# Autodesk Inventor assembly: Pool House 02
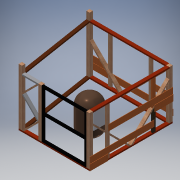
[picture p0: Inventor's stored thumbnail of the model, 180x180]
Saved by Autodesk Inventor 2016 (Build 200138000, 138)
## iProperties
Created: 2015-05-30
Part Number: Pool House 02
Document SubType Name: Assembly
Designer: steele
Author: steele
## Documents named in this file (28)
- C:\snobotics\CAD-Development\robSteele\HouseProjects\PoolHouseProject\Pool House 02.iam
- C:\snobotics\CAD-Development\robSteele\HouseProjects\PoolHouseProject\Base for Pool House.ipt
- C:\snobotics\CAD-Development\robSteele\HouseProjects\PoolHouseProject\Front Post North Side.ipt
- C:\snobotics\CAD-Development\robSteele\HouseProjects\PoolHouseProject\Front Post South Side.ipt
- C:\snobotics\CAD-Development\robSteele\HouseProjects\PoolHouseProject\Rear Post South Side.ipt
- C:\snobotics\CAD-Development\robSteele\HouseProjects\PoolHouseProject\Pool Controller.ipt
- C:\snobotics\CAD-Development\robSteele\HouseProjects\PoolHouseProject\Home Depot Composite Slat 69 in.ipt
- C:\snobotics\CAD-Development\robSteele\HouseProjects\PoolHouseProject\Home Depot Composite Slat 19_75 in.ipt
- C:\snobotics\CAD-Development\robSteele\HouseProjects\PoolHouseProject\Lumber 2x4x82.ipt
- C:\snobotics\CAD-Development\robSteele\HouseProjects\PoolHouseProject\Lumbwer 2x4x50_75.ipt
- C:\snobotics\CAD-Development\robSteele\HouseProjects\PoolHouseProject\Lumber 2x4x80.ipt
- C:\snobotics\CAD-Development\robSteele\HouseProjects\PoolHouseProject\Pool Filter.ipt
- C:\snobotics\CAD-Development\robSteele\HouseProjects\PoolHouseProject\Pool Door.ipt
- C:\snobotics\CAD-Development\robSteele\HouseProjects\PoolHouseProject\58 Inch 45 Diagonal Piece.ipt
- C:\snobotics\CAD-Development\robSteele\HouseProjects\PoolHouseProject\Roof.ipt
- C:\snobotics\CAD-Development\robSteele\HouseProjects\PoolHouseProject\Front Face Bottom Support for Slats.ipt
- C:\snobotics\CAD-Development\robSteele\HouseProjects\PoolHouseProject\Front Face Upper Support for Slats.ipt
- C:\snobotics\CAD-Development\robSteele\HouseProjects\PoolHouseProject\Right Panel Rear 45 Diagonal Piece.ipt
- C:\snobotics\CAD-Development\robSteele\HouseProjects\PoolHouseProject\New Rear Post North Side.ipt
- C:\snobotics\CAD-Development\robSteele\HouseProjects\PoolHouseProject\Right Panel Front 45 Diagonal Piece.ipt
- C:\snobotics\CAD-Development\robSteele\HouseProjects\PoolHouseProject\Back 2x4.ipt
- C:\snobotics\CAD-Development\robSteele\HouseProjects\PoolHouseProject\Support 2x4.ipt
- C:\snobotics\CAD-Development\robSteele\HouseProjects\PoolHouseProject\Home Depot Composite Slat 51_5 in.ipt
- C:\snobotics\CAD-Development\robSteele\HouseProjects\PoolHouseProject\2x4 17.5 Inch.ipt
- C:\snobotics\CAD-Development\robSteele\HouseProjects\PoolHouseProject\Short Wall 45 Diagonal Piece.ipt
- C:\snobotics\CAD-Development\robSteele\HouseProjects\PoolHouseProject\Home Depot Composite Slat 24_50 in.ipt
- C:\snobotics\CAD-Development\robSteele\HouseProjects\PoolHouseProject\Home Depot Composite Slat 23 in.ipt
- C:\snobotics\CAD-Development\robSteele\HouseProjects\PoolHouseProject\Home Depot Composite Slat 66 3_16 in.ipt
## Components (76 placed, 27 different names)
1. Base for Pool House:1 — Mate:1, Flush:1, Flush:2, Mate:2, Flush:3, Flush:4, Mate:3, Flush:5, Flush:6, Mate:4, Flush:7, Flush:8, Mate:8, Flush:11, Mate:9, Mate:10, Flush:21, Flush:22, Mate:77, Mate:79, Mate:82, Flush:32, Mate:84, Flush:33, Flush:34, Tangent:1, Tangent:2, Mate:93, Mate:100, Mate:102, Mate:112, Mate:114, Mate:115, Flush:47, Flush:48, Mate:116, Flush:49, Mate:117, Mate:119, Mate:127
2. Front Post North Side:1 — Mate:1, Flush:1, Flush:2, Mate:5, Flush:9, Flush:10, Mate:11, Mate:12, Mate:13, Mate:20, Mate:24, Mate:28, Mate:32, Mate:38, Mate:40, Mate:78, Flush:58, Flush:59, Flush:60, Flush:73
3. Front Post South Side:1 — Mate:2, Flush:3, Flush:4, Mate:7, Mate:15, Mate:22, Mate:27, Mate:30, Mate:34, Mate:36, Mate:42, Mate:80, Mate:81, Flush:30, Flush:31, Mate:85, Mate:94, Flush:38, Mate:101, Flush:40, Mate:104, Mate:108, Mate:111, Flush:45, Flush:74
4. Front Post North Side:3 — Mate:3, Flush:5, Flush:6, Mate:92, Mate:118, Flush:50, Flush:51, Mate:120
5. Rear Post South Side:1 — Mate:4, Flush:7, Flush:8, Mate:45, Mate:47, Mate:53, Mate:55, Mate:61, Mate:69, Mate:71, Mate:75, Mate:83, Mate:113, Flush:46
6. Pool Controller:1 — Mate:5, Flush:9, Flush:10
7. Lumber 2x4x82:1 — Mate:11, Mate:12, Mate:97
8. Home Depot Composite Slat 69 in:1 — Mate:7, Mate:8, Flush:11, Mate:16, Flush:14, Mate:46, Flush:61
9. Home Depot Composite Slat 19_75 in:1 — Mate:9, Mate:10, Mate:14, Flush:14
10. Home Depot Composite Slat 69 in:2 — Mate:13, Mate:14, Mate:21, Mate:23, Flush:13, Flush:60
11. Home Depot Composite Slat 19_75 in:2 — Mate:15, Mate:16, Flush:13, Mate:49
12. Home Depot Composite Slat 69 in:3 — Mate:22, Mate:23, Flush:12, Mate:26, Mate:51, Flush:62
13. Home Depot Composite Slat 19_75 in:3 — Mate:20, Mate:21, Flush:12, Mate:25
14. Home Depot Composite Slat 69 in:4 — Mate:24, Mate:25, Flush:15, Mate:29, Flush:59
15. Home Depot Composite Slat 19_75 in:4 — Mate:26, Mate:27, Flush:15, Mate:31, Mate:57
16. Home Depot Composite Slat 19_75 in:5 — Mate:28, Mate:29, Flush:16
17. Home Depot Composite Slat 69 in:5 — Mate:30, Mate:31, Flush:16, Mate:33, Mate:35, Mate:59, Flush:63
18. Home Depot Composite Slat 69 in:6 — Mate:32, Mate:33, Flush:17, Mate:39
19. Home Depot Composite Slat 19_75 in:6 — Mate:34, Mate:35, Flush:17, Mate:37, Flush:29, Flush:64
20. Home Depot Composite Slat 69 in:7 — Mate:36, Mate:37, Flush:18, Mate:41, Mate:43, Mate:65, Flush:29, Flush:65
21. Home Depot Composite Slat 19_75 in:7 — Mate:38, Mate:39, Flush:18
22. Home Depot Composite Slat 69 in:8 — Mate:40, Mate:41, Flush:19, Mate:148, Flush:58
23. Home Depot Composite Slat 19_75 in:8 — Mate:42, Mate:43, Flush:19, Mate:67, Mate:73
24. Home Depot Composite Slat 23 in:1 — Mate:45, Flush:21, Mate:48, Flush:23
25. Home Depot Composite Slat 66 3_16 in:1 — Mate:46, Flush:22, Flush:23, Mate:50, Flush:61
26. Home Depot Composite Slat 66 3_16 in:2 — Mate:47, Mate:48, Flush:24, Mate:54
27. Home Depot Composite Slat 23 in:8 — Mate:49, Mate:50, Flush:24, Mate:52
28. Home Depot Composite Slat 66 3_16 in:3 — Mate:51, Mate:52, Flush:25, Mate:58, Flush:62
29. Home Depot Composite Slat 23 in:4 — Mate:53, Mate:54, Flush:25, Mate:56
30. Home Depot Composite Slat 66 3_16 in:8 — Mate:55, Mate:56, Flush:26, Mate:62
31. Home Depot Composite Slat 23 in:5 — Mate:57, Mate:58, Flush:26, Mate:60
32. Home Depot Composite Slat 66 3_16 in:7 — Mate:59, Mate:60, Flush:27, Mate:64, Mate:70, Flush:63
33. Home Depot Composite Slat 66 3_16 in:5 — Mate:64, Mate:69, Flush:28, Mate:72
34. Home Depot Composite Slat 66 3_16 in:6 — Mate:67, Mate:68, Mate:74, Mate:76, Flush:65
35. Home Depot Composite Slat 23 in:2 — Mate:61, Mate:62, Flush:27
36. Home Depot Composite Slat 23 in:6 — Mate:65, Mate:68, Mate:70, Flush:28, Flush:64
37. Home Depot Composite Slat 23 in:7 — Mate:71, Mate:72
38. Home Depot Composite Slat 23 in:3 — Mate:73, Mate:74, Mate:151
39. Home Depot Composite Slat 66 3_16 in:4 — Mate:75, Mate:76
40. Lumbwer 2x4x50_75:1 — Mate:77, Mate:78, Mate:148
41. Lumbwer 2x4x50_75:2 — Mate:79, Mate:80
42. Lumber 2x4x80:1 — Mate:81, Flush:30, Flush:31
43. Lumbwer 2x4x50_75:3 — Mate:82, Mate:83, Flush:32
44. Lumbwer 2x4x50_75:4 — Mate:84, Mate:85, Flush:33, Mate:151
45. Pool Filter:1 — Flush:34, Tangent:1, Tangent:2
46. Pool Door:1 — Mate:92, Mate:93, Mate:146, Mate:147, Flush:57, Mate:153, Flush:66, Mate:155, Flush:67, Mate:157, Flush:68, Mate:159, Flush:69, Mate:161, Flush:70, Mate:163, Flush:71, Mate:165, Flush:72
47. 58 Inch 45 Diagonal Piece:1 — Mate:100, Flush:73
48. 58 Inch 45 Diagonal Piece:2 — Mate:94, Flush:38, Mate:97, Mate:101, Mate:102, Flush:40, Mate:103, Flush:41, Mate:107, Flush:42, Flush:74
49. Roof:1
50. Front Face Bottom Support for Slats:1 — Mate:103, Mate:104, Flush:41
51. Front Face Upper Support for Slats:2 — Mate:107, Mate:108, Flush:42
52. Right Panel Front 45 Diagonal Piece:1 — Mate:111, Mate:112, Flush:45
53. Right Panel Rear 45 Diagonal Piece:2 — Mate:113, Mate:114, Flush:46
54. New Rear Post North Side:1 — Mate:115, Flush:47, Flush:48, Flush:52, Mate:122, Flush:53, Mate:123, Mate:124, Mate:128, Mate:129, Mate:132, Mate:133, Mate:134, Mate:136, Mate:138, Mate:140, Mate:142
55. Back 2x4:1 — Mate:116, Flush:49, Mate:117
56. 2x4 17.5 Inch:1 — Mate:118, Flush:50, Flush:51, Mate:121, Flush:54
57. Short Wall 45 Diagonal Piece:2 — Mate:119, Mate:120, Flush:52
58. Short Wall 45 Diagonal Piece:1 — Mate:121, Mate:122, Flush:53, Flush:56, Mate:149, Mate:150
59. Back 2x4:2 — Mate:123, Flush:54, Mate:124
60. Home Depot Composite Slat 24_50 in:1 — Mate:127, Mate:128, Mate:130
61. Home Depot Composite Slat 24_50 in:2 — Mate:129, Mate:130, Mate:131
62. Home Depot Composite Slat 24_50 in:3 — Mate:131, Mate:132, Mate:135
63. Home Depot Composite Slat 24_50 in:4 — Mate:133, Mate:134, Mate:135, Mate:137
64. Home Depot Composite Slat 24_50 in:5 — Mate:136, Mate:137, Mate:139
65. Home Depot Composite Slat 24_50 in:6 — Mate:138, Mate:139, Mate:141
66. Home Depot Composite Slat 24_50 in:7 — Mate:140, Mate:141, Mate:143
67. Home Depot Composite Slat 24_50 in:8 — Mate:142, Mate:143
68. Support 2x4:1 — Flush:56, Mate:149, Mate:150
69. Home Depot Composite Slat 51_5 in:1 — Mate:146, Mate:147, Flush:57, Mate:152
70. Home Depot Composite Slat 51_5 in:2 — Mate:152, Mate:153, Flush:66, Mate:154
71. Home Depot Composite Slat 51_5 in:3 — Mate:154, Mate:155, Flush:67, Mate:156
72. Home Depot Composite Slat 51_5 in:4 — Mate:156, Mate:157, Flush:68, Mate:158
73. Home Depot Composite Slat 51_5 in:5 — Mate:158, Mate:159, Flush:69, Mate:160
74. Home Depot Composite Slat 51_5 in:6 — Mate:160, Mate:161, Flush:70, Mate:162
75. Home Depot Composite Slat 51_5 in:7 — Mate:162, Mate:163, Flush:71, Mate:164
76. Home Depot Composite Slat 51_5 in:8 — Mate:164, Mate:165, Flush:72
## Relationships (208: Mate 140, Flush 66, Tangent 2)
- Mate:1: Base for Pool House:1 ↔ Front Post North Side:1
- Flush:1: Base for Pool House:1 ↔ Front Post North Side:1
- Flush:2: Base for Pool House:1 ↔ Front Post North Side:1
- Mate:2: Base for Pool House:1 ↔ Front Post South Side:1
- Flush:3: Base for Pool House:1 ↔ Front Post South Side:1
- Flush:4: Base for Pool House:1 ↔ Front Post South Side:1
- Mate:3: Base for Pool House:1 ↔ Front Post North Side:3
- Flush:5: Base for Pool House:1 ↔ Front Post North Side:3
- Flush:6 (533.4 mm): Base for Pool House:1 ↔ Front Post North Side:3
- Mate:4: Base for Pool House:1 ↔ Rear Post South Side:1
- Flush:7: Base for Pool House:1 ↔ Rear Post South Side:1
- Flush:8: Base for Pool House:1 ↔ Rear Post South Side:1
- Mate:5 (127 mm): Front Post North Side:1 ↔ Pool Controller:1
- Flush:9 (120.65 mm): Front Post North Side:1 ↔ Pool Controller:1
- Flush:10 (101.6 mm): Front Post North Side:1 ↔ Pool Controller:1
- Mate:7: Front Post South Side:1 ↔ Home Depot Composite Slat 69 in:1
- Mate:8: Base for Pool House:1 ↔ Home Depot Composite Slat 69 in:1
- Flush:11: Base for Pool House:1 ↔ Home Depot Composite Slat 69 in:1
- Mate:9: Base for Pool House:1 ↔ Home Depot Composite Slat 19_75 in:1
- Mate:10: Base for Pool House:1 ↔ Home Depot Composite Slat 19_75 in:1
- Mate:11: Front Post North Side:1 ↔ Lumber 2x4x82:1
- Mate:12: Front Post North Side:1 ↔ Lumber 2x4x82:1
- Mate:13: Front Post North Side:1 ↔ Home Depot Composite Slat 69 in:2
- Mate:14 (6.35 mm): Home Depot Composite Slat 19_75 in:1 ↔ Home Depot Composite Slat 69 in:2
- Mate:15: Front Post South Side:1 ↔ Home Depot Composite Slat 19_75 in:2
- Mate:16 (6.35 mm): Home Depot Composite Slat 69 in:1 ↔ Home Depot Composite Slat 19_75 in:2
- Mate:20: Front Post North Side:1 ↔ Home Depot Composite Slat 19_75 in:3
- Mate:21 (6.35 mm): Home Depot Composite Slat 69 in:2 ↔ Home Depot Composite Slat 19_75 in:3
- Mate:22: Front Post South Side:1 ↔ Home Depot Composite Slat 69 in:3
- Mate:23 (6.35 mm): Home Depot Composite Slat 69 in:2 ↔ Home Depot Composite Slat 69 in:3
- Flush:12: Home Depot Composite Slat 69 in:3 ↔ Home Depot Composite Slat 19_75 in:3
- Flush:13: Home Depot Composite Slat 69 in:2 ↔ Home Depot Composite Slat 19_75 in:2
- Flush:14: Home Depot Composite Slat 69 in:1 ↔ Home Depot Composite Slat 19_75 in:1
- Mate:24: Front Post North Side:1 ↔ Home Depot Composite Slat 69 in:4
- Mate:25 (6.35 mm): Home Depot Composite Slat 19_75 in:3 ↔ Home Depot Composite Slat 69 in:4
- Mate:26 (6.35 mm): Home Depot Composite Slat 69 in:3 ↔ Home Depot Composite Slat 19_75 in:4
- Mate:27: Front Post South Side:1 ↔ Home Depot Composite Slat 19_75 in:4
- Flush:15: Home Depot Composite Slat 69 in:4 ↔ Home Depot Composite Slat 19_75 in:4
- Mate:28: Front Post North Side:1 ↔ Home Depot Composite Slat 19_75 in:5
- Mate:29 (6.35 mm): Home Depot Composite Slat 69 in:4 ↔ Home Depot Composite Slat 19_75 in:5
- Mate:30: Front Post South Side:1 ↔ Home Depot Composite Slat 69 in:5
- Mate:31 (6.35 mm): Home Depot Composite Slat 19_75 in:4 ↔ Home Depot Composite Slat 69 in:5
- Flush:16: Home Depot Composite Slat 19_75 in:5 ↔ Home Depot Composite Slat 69 in:5
- Mate:32: Front Post North Side:1 ↔ Home Depot Composite Slat 69 in:6
- Mate:33 (6.35 mm): Home Depot Composite Slat 69 in:5 ↔ Home Depot Composite Slat 69 in:6
- Mate:34: Front Post South Side:1 ↔ Home Depot Composite Slat 19_75 in:6
- Mate:35 (6.35 mm): Home Depot Composite Slat 69 in:5 ↔ Home Depot Composite Slat 19_75 in:6
- Flush:17: Home Depot Composite Slat 69 in:6 ↔ Home Depot Composite Slat 19_75 in:6
- Mate:36: Front Post South Side:1 ↔ Home Depot Composite Slat 69 in:7
- Mate:37 (6.35 mm): Home Depot Composite Slat 19_75 in:6 ↔ Home Depot Composite Slat 69 in:7
- Mate:38: Front Post North Side:1 ↔ Home Depot Composite Slat 19_75 in:7
- Mate:39 (6.35 mm): Home Depot Composite Slat 69 in:6 ↔ Home Depot Composite Slat 19_75 in:7
- Flush:18: Home Depot Composite Slat 69 in:7 ↔ Home Depot Composite Slat 19_75 in:7
- Mate:40: Front Post North Side:1 ↔ Home Depot Composite Slat 69 in:8
- Mate:41 (6.35 mm): Home Depot Composite Slat 69 in:7 ↔ Home Depot Composite Slat 69 in:8
- Mate:42: Front Post South Side:1 ↔ Home Depot Composite Slat 19_75 in:8
- Mate:43 (6.35 mm): Home Depot Composite Slat 69 in:7 ↔ Home Depot Composite Slat 19_75 in:8
- Flush:19: Home Depot Composite Slat 69 in:8 ↔ Home Depot Composite Slat 19_75 in:8
- Mate:45: Rear Post South Side:1 ↔ Home Depot Composite Slat 23 in:1
- Flush:21: Base for Pool House:1 ↔ Home Depot Composite Slat 23 in:1
- Mate:46: Home Depot Composite Slat 69 in:1 ↔ Home Depot Composite Slat 66 3_16 in:1
- Flush:22: Base for Pool House:1 ↔ Home Depot Composite Slat 66 3_16 in:1
- Mate:47: Rear Post South Side:1 ↔ Home Depot Composite Slat 66 3_16 in:2
- Mate:48 (6.35 mm): Home Depot Composite Slat 23 in:1 ↔ Home Depot Composite Slat 66 3_16 in:2
- Flush:23: Home Depot Composite Slat 23 in:1 ↔ Home Depot Composite Slat 66 3_16 in:1
- Mate:49: Home Depot Composite Slat 19_75 in:2 ↔ Home Depot Composite Slat 23 in:8
- Mate:50 (6.35 mm): Home Depot Composite Slat 66 3_16 in:1 ↔ Home Depot Composite Slat 23 in:8
- Flush:24: Home Depot Composite Slat 66 3_16 in:2 ↔ Home Depot Composite Slat 23 in:8
- Mate:51: Home Depot Composite Slat 69 in:3 ↔ Home Depot Composite Slat 66 3_16 in:3
- Mate:52 (6.35 mm): Home Depot Composite Slat 23 in:8 ↔ Home Depot Composite Slat 66 3_16 in:3
- Mate:53: Rear Post South Side:1 ↔ Home Depot Composite Slat 23 in:4
- Mate:54 (6.35 mm): Home Depot Composite Slat 66 3_16 in:2 ↔ Home Depot Composite Slat 23 in:4
- Flush:25: Home Depot Composite Slat 66 3_16 in:3 ↔ Home Depot Composite Slat 23 in:4
- Mate:55: Rear Post South Side:1 ↔ Home Depot Composite Slat 66 3_16 in:8
- Mate:56 (6.35 mm): Home Depot Composite Slat 23 in:4 ↔ Home Depot Composite Slat 66 3_16 in:8
- Mate:57: Home Depot Composite Slat 19_75 in:4 ↔ Home Depot Composite Slat 23 in:5
- Mate:58 (6.35 mm): Home Depot Composite Slat 66 3_16 in:3 ↔ Home Depot Composite Slat 23 in:5
- Flush:26: Home Depot Composite Slat 66 3_16 in:8 ↔ Home Depot Composite Slat 23 in:5
- Mate:59: Home Depot Composite Slat 69 in:5 ↔ Home Depot Composite Slat 66 3_16 in:7
- Mate:60 (6.35 mm): Home Depot Composite Slat 23 in:5 ↔ Home Depot Composite Slat 66 3_16 in:7
- Mate:61: Rear Post South Side:1 ↔ Home Depot Composite Slat 23 in:2
- Mate:62 (6.35 mm): Home Depot Composite Slat 66 3_16 in:8 ↔ Home Depot Composite Slat 23 in:2
- Flush:27: Home Depot Composite Slat 66 3_16 in:7 ↔ Home Depot Composite Slat 23 in:2
- Mate:64 (6.35 mm): Home Depot Composite Slat 66 3_16 in:7 ↔ Home Depot Composite Slat 66 3_16 in:5
- Mate:65: Home Depot Composite Slat 69 in:7 ↔ Home Depot Composite Slat 23 in:6
- Mate:67: Home Depot Composite Slat 19_75 in:8 ↔ Home Depot Composite Slat 66 3_16 in:6
- Mate:68 (6.35 mm): Home Depot Composite Slat 66 3_16 in:6 ↔ Home Depot Composite Slat 23 in:6
- Mate:69: Rear Post South Side:1 ↔ Home Depot Composite Slat 66 3_16 in:5
- Mate:70 (6.35 mm): Home Depot Composite Slat 66 3_16 in:7 ↔ Home Depot Composite Slat 23 in:6
- Flush:28: Home Depot Composite Slat 66 3_16 in:5 ↔ Home Depot Composite Slat 23 in:6
- Flush:29: Home Depot Composite Slat 19_75 in:6 ↔ Home Depot Composite Slat 69 in:7
- Mate:71: Rear Post South Side:1 ↔ Home Depot Composite Slat 23 in:7
- Mate:72 (6.35 mm): Home Depot Composite Slat 66 3_16 in:5 ↔ Home Depot Composite Slat 23 in:7
- Mate:73: Home Depot Composite Slat 19_75 in:8 ↔ Home Depot Composite Slat 23 in:3
- Mate:74 (6.35 mm): Home Depot Composite Slat 66 3_16 in:6 ↔ Home Depot Composite Slat 23 in:3
- Mate:75: Rear Post South Side:1 ↔ Home Depot Composite Slat 66 3_16 in:4
- Mate:76 (6.35 mm): Home Depot Composite Slat 66 3_16 in:6 ↔ Home Depot Composite Slat 66 3_16 in:4
- Mate:77: Base for Pool House:1 ↔ Lumbwer 2x4x50_75:1
- Mate:78 (371.475 mm): Front Post North Side:1 ↔ Lumbwer 2x4x50_75:1
- Mate:79: Base for Pool House:1 ↔ Lumbwer 2x4x50_75:2
- Mate:80 (371.475 mm): Front Post South Side:1 ↔ Lumbwer 2x4x50_75:2
- Mate:81: Front Post South Side:1 ↔ Lumber 2x4x80:1
- Flush:30: Front Post South Side:1 ↔ Lumber 2x4x80:1
- Flush:31: Front Post South Side:1 ↔ Lumber 2x4x80:1
- Mate:82: Base for Pool House:1 ↔ Lumbwer 2x4x50_75:3
- Mate:83 (450.8373 mm): Rear Post South Side:1 ↔ Lumbwer 2x4x50_75:3
- Flush:32: Base for Pool House:1 ↔ Lumbwer 2x4x50_75:3
- Mate:84: Base for Pool House:1 ↔ Lumbwer 2x4x50_75:4
- Mate:85 (436.4355 mm): Front Post South Side:1 ↔ Lumbwer 2x4x50_75:4
- Flush:33: Base for Pool House:1 ↔ Lumbwer 2x4x50_75:4
- Flush:34: Base for Pool House:1 ↔ Pool Filter:1
- Tangent:1 (609.6 mm): Base for Pool House:1 ↔ Pool Filter:1
- Tangent:2 (609.6 mm): Base for Pool House:1 ↔ Pool Filter:1
- Mate:92: Front Post North Side:3 ↔ Pool Door:1
- Mate:93: Base for Pool House:1 ↔ Pool Door:1
- Mate:94: Front Post South Side:1 ↔ 58 Inch 45 Diagonal Piece:2
- Flush:38: Front Post South Side:1 ↔ 58 Inch 45 Diagonal Piece:2
- Mate:97 (254 mm): Lumber 2x4x82:1 ↔ 58 Inch 45 Diagonal Piece:2
- Mate:100: Base for Pool House:1 ↔ 58 Inch 45 Diagonal Piece:1
- Mate:101: Front Post South Side:1 ↔ 58 Inch 45 Diagonal Piece:2
- Mate:102: Base for Pool House:1 ↔ 58 Inch 45 Diagonal Piece:2
- Flush:40: Front Post South Side:1 ↔ 58 Inch 45 Diagonal Piece:2
- Mate:103: 58 Inch 45 Diagonal Piece:2 ↔ Front Face Bottom Support for Slats:1
- Mate:104 (371.475 mm): Front Post South Side:1 ↔ Front Face Bottom Support for Slats:1
- Flush:41: 58 Inch 45 Diagonal Piece:2 ↔ Front Face Bottom Support for Slats:1
- Mate:107: 58 Inch 45 Diagonal Piece:2 ↔ Front Face Upper Support for Slats:2
- Mate:108 (371.475 mm): Front Post South Side:1 ↔ Front Face Upper Support for Slats:2
- Flush:42: 58 Inch 45 Diagonal Piece:2 ↔ Front Face Upper Support for Slats:2
- Mate:111: Front Post South Side:1 ↔ Right Panel Front 45 Diagonal Piece:1
- Mate:112: Base for Pool House:1 ↔ Right Panel Front 45 Diagonal Piece:1
- Flush:45: Front Post South Side:1 ↔ Right Panel Front 45 Diagonal Piece:1
- Mate:113: Rear Post South Side:1 ↔ Right Panel Rear 45 Diagonal Piece:2
- Mate:114: Base for Pool House:1 ↔ Right Panel Rear 45 Diagonal Piece:2
- Flush:46: Rear Post South Side:1 ↔ Right Panel Rear 45 Diagonal Piece:2
- Mate:115: Base for Pool House:1 ↔ New Rear Post North Side:1
- Flush:47: Base for Pool House:1 ↔ New Rear Post North Side:1
- Flush:48: Base for Pool House:1 ↔ New Rear Post North Side:1
- Mate:116: Base for Pool House:1 ↔ Back 2x4:1
- Flush:49: Base for Pool House:1 ↔ Back 2x4:1
- Mate:117: Base for Pool House:1 ↔ Back 2x4:1
- Mate:118: Front Post North Side:3 ↔ 2x4 17.5 Inch:1
- Flush:50: Front Post North Side:3 ↔ 2x4 17.5 Inch:1
- Flush:51: Front Post North Side:3 ↔ 2x4 17.5 Inch:1
- Mate:119: Base for Pool House:1 ↔ Short Wall 45 Diagonal Piece:2
- Mate:120: Front Post North Side:3 ↔ Short Wall 45 Diagonal Piece:2
- Flush:52: New Rear Post North Side:1 ↔ Short Wall 45 Diagonal Piece:2
- Mate:121: 2x4 17.5 Inch:1 ↔ Short Wall 45 Diagonal Piece:1
- Mate:122: New Rear Post North Side:1 ↔ Short Wall 45 Diagonal Piece:1
- Flush:53: New Rear Post North Side:1 ↔ Short Wall 45 Diagonal Piece:1
- Mate:123: New Rear Post North Side:1 ↔ Back 2x4:2
- Flush:54: 2x4 17.5 Inch:1 ↔ Back 2x4:2
- Mate:124: New Rear Post North Side:1 ↔ Back 2x4:2
- Mate:127: Base for Pool House:1 ↔ Home Depot Composite Slat 24_50 in:1
- Mate:128: New Rear Post North Side:1 ↔ Home Depot Composite Slat 24_50 in:1
- Mate:129: New Rear Post North Side:1 ↔ Home Depot Composite Slat 24_50 in:2
- Mate:130 (6.35 mm): Home Depot Composite Slat 24_50 in:1 ↔ Home Depot Composite Slat 24_50 in:2
- Mate:131 (6.35 mm): Home Depot Composite Slat 24_50 in:2 ↔ Home Depot Composite Slat 24_50 in:3
- Mate:132: New Rear Post North Side:1 ↔ Home Depot Composite Slat 24_50 in:3
- Mate:133: New Rear Post North Side:1 ↔ Home Depot Composite Slat 24_50 in:4
- Mate:134: New Rear Post North Side:1 ↔ Home Depot Composite Slat 24_50 in:4
- Mate:135 (6.35 mm): Home Depot Composite Slat 24_50 in:3 ↔ Home Depot Composite Slat 24_50 in:4
- Mate:136: New Rear Post North Side:1 ↔ Home Depot Composite Slat 24_50 in:5
- Mate:137 (6.35 mm): Home Depot Composite Slat 24_50 in:4 ↔ Home Depot Composite Slat 24_50 in:5
- Mate:138: New Rear Post North Side:1 ↔ Home Depot Composite Slat 24_50 in:6
- Mate:139 (6.35 mm): Home Depot Composite Slat 24_50 in:5 ↔ Home Depot Composite Slat 24_50 in:6
- Mate:140: New Rear Post North Side:1 ↔ Home Depot Composite Slat 24_50 in:7
- Mate:141 (6.35 mm): Home Depot Composite Slat 24_50 in:6 ↔ Home Depot Composite Slat 24_50 in:7
- Mate:142: New Rear Post North Side:1 ↔ Home Depot Composite Slat 24_50 in:8
- Mate:143 (6.35 mm): Home Depot Composite Slat 24_50 in:7 ↔ Home Depot Composite Slat 24_50 in:8
- Flush:56: Short Wall 45 Diagonal Piece:1 ↔ Support 2x4:1
- Mate:146 (38.1 mm): Pool Door:1 ↔ Home Depot Composite Slat 51_5 in:1
- Mate:147: Pool Door:1 ↔ Home Depot Composite Slat 51_5 in:1
- Flush:57: Pool Door:1 ↔ Home Depot Composite Slat 51_5 in:1
- Mate:148: Home Depot Composite Slat 69 in:8 ↔ Lumbwer 2x4x50_75:1
- Flush:58: Front Post North Side:1 ↔ Home Depot Composite Slat 69 in:8
- Flush:59: Front Post North Side:1 ↔ Home Depot Composite Slat 69 in:4
- Flush:60: Front Post North Side:1 ↔ Home Depot Composite Slat 69 in:2
- Mate:149: Short Wall 45 Diagonal Piece:1 ↔ Support 2x4:1
- Mate:150: Short Wall 45 Diagonal Piece:1 ↔ Support 2x4:1
- Mate:151: Home Depot Composite Slat 23 in:3 ↔ Lumbwer 2x4x50_75:4
- Flush:61: Home Depot Composite Slat 69 in:1 ↔ Home Depot Composite Slat 66 3_16 in:1
- Flush:62: Home Depot Composite Slat 69 in:3 ↔ Home Depot Composite Slat 66 3_16 in:3
- Flush:63: Home Depot Composite Slat 69 in:5 ↔ Home Depot Composite Slat 66 3_16 in:7
- Flush:64: Home Depot Composite Slat 19_75 in:6 ↔ Home Depot Composite Slat 23 in:6
- Flush:65: Home Depot Composite Slat 69 in:7 ↔ Home Depot Composite Slat 66 3_16 in:6
- Mate:152 (6.35 mm): Home Depot Composite Slat 51_5 in:1 ↔ Home Depot Composite Slat 51_5 in:2
- Mate:153: Pool Door:1 ↔ Home Depot Composite Slat 51_5 in:2
- Flush:66: Pool Door:1 ↔ Home Depot Composite Slat 51_5 in:2
- Mate:154 (6.35 mm): Home Depot Composite Slat 51_5 in:2 ↔ Home Depot Composite Slat 51_5 in:3
- Mate:155: Pool Door:1 ↔ Home Depot Composite Slat 51_5 in:3
- Flush:67: Pool Door:1 ↔ Home Depot Composite Slat 51_5 in:3
- Mate:156 (6.35 mm): Home Depot Composite Slat 51_5 in:3 ↔ Home Depot Composite Slat 51_5 in:4
- Mate:157: Pool Door:1 ↔ Home Depot Composite Slat 51_5 in:4
- Flush:68: Pool Door:1 ↔ Home Depot Composite Slat 51_5 in:4
- Mate:158 (6.35 mm): Home Depot Composite Slat 51_5 in:4 ↔ Home Depot Composite Slat 51_5 in:5
- Mate:159: Pool Door:1 ↔ Home Depot Composite Slat 51_5 in:5
- Flush:69: Pool Door:1 ↔ Home Depot Composite Slat 51_5 in:5
- Mate:160 (6.35 mm): Home Depot Composite Slat 51_5 in:5 ↔ Home Depot Composite Slat 51_5 in:6
- Mate:161: Pool Door:1 ↔ Home Depot Composite Slat 51_5 in:6
- Flush:70: Pool Door:1 ↔ Home Depot Composite Slat 51_5 in:6
- Mate:162 (6.35 mm): Home Depot Composite Slat 51_5 in:6 ↔ Home Depot Composite Slat 51_5 in:7
- Mate:163: Pool Door:1 ↔ Home Depot Composite Slat 51_5 in:7
- Flush:71: Pool Door:1 ↔ Home Depot Composite Slat 51_5 in:7
- Mate:164 (6.35 mm): Home Depot Composite Slat 51_5 in:7 ↔ Home Depot Composite Slat 51_5 in:8
- Mate:165: Pool Door:1 ↔ Home Depot Composite Slat 51_5 in:8
- Flush:72: Pool Door:1 ↔ Home Depot Composite Slat 51_5 in:8
- Flush:73: Front Post North Side:1 ↔ 58 Inch 45 Diagonal Piece:1
- Flush:74: Front Post South Side:1 ↔ 58 Inch 45 Diagonal Piece:2
